# Autodesk Inventor assembly: Ensamble
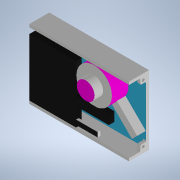
[picture p0: Inventor's stored thumbnail of the model, 180x180]
Saved by Autodesk Inventor 2021 (Build 250183000, 183)
## iProperties
Created: 2021-02-21
Part Number: Ensamble
Document SubType Name: Assembly
Designer: deuts
Author: deuts
## Documents named in this file (5)
- C:\Users\deuts\Desktop\Mateus\Ensamble.iam
- C:\Users\deuts\Desktop\Mateus\Camara.ipt
- C:\Users\deuts\Desktop\Mateus\NVidia.ipt
- C:\Users\deuts\Desktop\Mateus\Caja1.ipt
- C:\Users\deuts\Desktop\Mateus\Caja2.ipt
## Components (4 placed, 4 different names)
1. Camara:1 — Flush:1, Angle:1, Flush:4
2. NVidia:1 — Flush:1, Angle:1, Mate:1, Flush:2, Flush:3
3. Caja1:1 — Mate:1, Flush:2, Flush:3, Flush:4, Mate:2
4. Caja2:1 — Mate:2
## Relationships (7: Flush 4, Mate 2, Angle 1)
- Flush:1: Camara:1 ↔ NVidia:1
- Angle:1 (135 deg): Camara:1 ↔ NVidia:1
- Mate:1: NVidia:1 ↔ Caja1:1
- Flush:2: NVidia:1 ↔ Caja1:1
- Flush:3: NVidia:1 ↔ Caja1:1
- Flush:4: Camara:1 ↔ Caja1:1
- Mate:2: Caja1:1 ↔ Caja2:1
